# Autodesk Inventor assembly: MG-Dribblingwelle
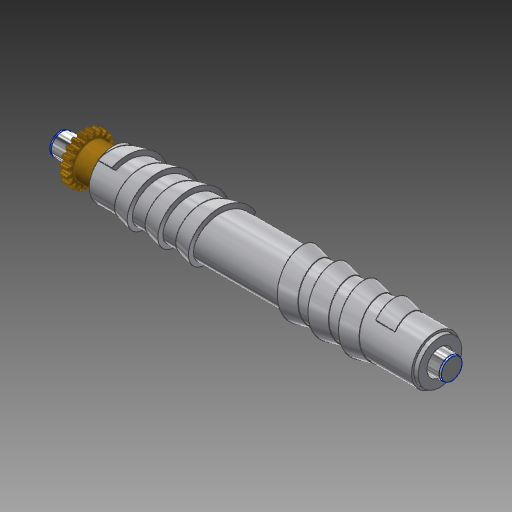
[picture p0: Inventor's stored thumbnail of the model, 512x512]
Saved by Autodesk Inventor 2019.4 (Build 234330000, 330)
## iProperties
Part Number: MG-Dribblingwelle
Material: Generisch
Document SubType Name: Assembly
Designer: rYan
Mass: 18.1168 g
Surface Area: 67.7067 cm^2
Volume: 8.51895 cm^3
Density: 2.12665 g/cm^3
Author: rYan
## Documents named in this file (4)
- D:\TIGERsGIT\Hardware\mechanik\2020\Inventor\Robot\Dribbler\MG-Dribblingwelle.iam
- D:\TIGERsGIT\Hardware\mechanik\2020\Inventor\Robot\Dribbler\Dribblingwelle.ipt
- D:\TIGERsGIT\Hardware\mechanik\2020\Inventor\Robot\Dribbler\Dribblerschnecke.ipt
- D:\TIGERsGIT\Hardware\mechanik\2020\Inventor\Purchased Parts\Zahnrad Messing z20 Schnecke.ipt
## Components (3 placed, 3 different names)
1. Dribblingwelle:1 — Passend:2, Fluchtend:1, Einfügen:3
2. Dribblerschnecke:1 — Passend:2, Fluchtend:1
3. Zahnrad Messing z20 Schnecke:1 — Einfügen:3
## Relationships (3: Mate 1, Flush 1, Insert 1)
- Passend:2 [Mate]: Dribblingwelle:1 ↔ Dribblerschnecke:1
- Fluchtend:1 [Flush]: Dribblingwelle:1 ↔ Dribblerschnecke:1
- Einfügen:3 [Insert]: Dribblingwelle:1 ↔ Zahnrad Messing z20 Schnecke:1
